# Autodesk Inventor assembly: REAR ASSEMBLY
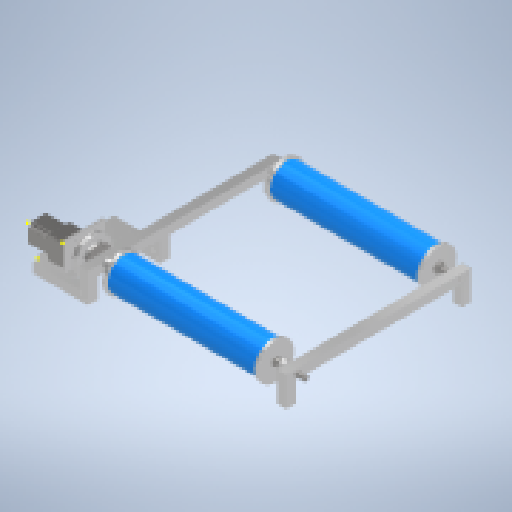
[picture p0: Inventor's stored thumbnail of the model, 512x512]
Saved by Autodesk Inventor 2023 (Build 270158000, 158)
## iProperties
Created: 2022-08-29
Part Number: REAR ASSEMBLY
Document SubType Name: Assembly
Designer: D.C. Eksteen
Author: D.C. Eksteen
## Documents named in this file (9)
- C:\Users\dylan\Desktop\Skripsie-2022\Design\CAD\REAR ASSEMBLY.iam
- C:\Users\dylan\Desktop\Skripsie-2022\Design\CAD\IDLE ROLLER.iam
- C:\Users\dylan\Desktop\Skripsie-2022\Design\CAD\POWER SHAFT ASSEMBLY.iam
- C:\Users\dylan\Desktop\Skripsie-2022\Design\CAD\LEFT FRAME.iam
- C:\Users\dylan\Desktop\Skripsie-2022\Design\CAD\RIGHT FRAME.iam
- C:\Users\dylan\Desktop\Skripsie-2022\Design\CAD\MOTOR MODEL.ipt
- C:\Users\dylan\Desktop\Skripsie-2022\Design\CAD\MOTOR BRACKET.ipt
- C:\Users\dylan\Desktop\Skripsie-2022\Design\CAD\ROTATING MAGNET DISC.ipt
- C:\Users\dylan\Desktop\Skripsie-2022\Design\CAD\METAL BACKPLATE.ipt
## Components (11 placed, 8 different names)
1. POWER SHAFT ASSEMBLY:1 [sub-assembly] — Mate:12, Mate:29
2. RIGHT FRAME:2 [sub-assembly]
3. LEFT FRAME:3 [sub-assembly] — Mate:13, Mate:19, Mate:20, Mate:21, Mate:22, Mate:23, Mate:24, Mate:30
4. IDLE ROLLER:1 [sub-assembly]
5. MOTOR MODEL:1 — Mate:15, Flush:1, Mate:30, Angle:1
6. MOTOR BRACKET:1 — Mate:12, Mate:13, Mate:15, Angle:1
7. ROTATING MAGNET DISC:1 — Mate:17, Mate:18, Mate:25, Mate:26, Mate:27, Mate:28, Flush:1, Mate:29
8. METAL BACKPLATE:1 — Mate:20, Mate:23, Mate:24
9. METAL BACKPLATE:2 — Mate:19, Mate:21, Mate:22
10. METAL BACKPLATE:3 — Mate:18, Mate:27, Mate:28
11. METAL BACKPLATE:4 — Mate:17, Mate:25, Mate:26
## Relationships (26: Mate 24, Flush 1, Angle 1)
- [Mate]: POWER SHAFT ASSEMBLY:1 ↔ RIGHT FRAME:2
- [Mate]: POWER SHAFT ASSEMBLY:1 ↔ RIGHT FRAME:2
- [Mate]: LEFT FRAME:3 ↔ IDLE ROLLER:1
- [Mate]: RIGHT FRAME:2 ↔ IDLE ROLLER:1
- [Mate]: LEFT FRAME:3 ↔ IDLE ROLLER:1
- [Mate]: RIGHT FRAME:2 ↔ IDLE ROLLER:1
- [Mate]: POWER SHAFT ASSEMBLY:1 ↔ LEFT FRAME:3
- Mate:12: POWER SHAFT ASSEMBLY:1 ↔ MOTOR BRACKET:1
- Mate:13: LEFT FRAME:3 ↔ MOTOR BRACKET:1
- Mate:15: MOTOR MODEL:1 ↔ MOTOR BRACKET:1
- Mate:17: ROTATING MAGNET DISC:1 ↔ METAL BACKPLATE:4
- Mate:18: ROTATING MAGNET DISC:1 ↔ METAL BACKPLATE:3
- Mate:19: LEFT FRAME:3 ↔ METAL BACKPLATE:2
- Mate:20: LEFT FRAME:3 ↔ METAL BACKPLATE:1
- Mate:21: LEFT FRAME:3 ↔ METAL BACKPLATE:2
- Mate:22: LEFT FRAME:3 ↔ METAL BACKPLATE:2
- Mate:23: LEFT FRAME:3 ↔ METAL BACKPLATE:1
- Mate:24: LEFT FRAME:3 ↔ METAL BACKPLATE:1
- Mate:25: ROTATING MAGNET DISC:1 ↔ METAL BACKPLATE:4
- Mate:26: ROTATING MAGNET DISC:1 ↔ METAL BACKPLATE:4
- Mate:27: ROTATING MAGNET DISC:1 ↔ METAL BACKPLATE:3
- Mate:28: ROTATING MAGNET DISC:1 ↔ METAL BACKPLATE:3
- Flush:1: MOTOR MODEL:1 ↔ ROTATING MAGNET DISC:1
- Mate:29 (3 mm): POWER SHAFT ASSEMBLY:1 ↔ ROTATING MAGNET DISC:1
- Mate:30: LEFT FRAME:3 ↔ MOTOR MODEL:1
- Angle:1 (0 deg): MOTOR MODEL:1 ↔ MOTOR BRACKET:1
